# Autodesk Inventor assembly: assembly_camera
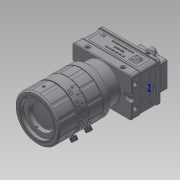
[picture p0: Inventor's stored thumbnail of the model, 180x180]
Saved by Autodesk Inventor 2017 (Build 210142000, 142)
## iProperties
Part Number: assembly_camera
Material: Generisch
Document SubType Name: Assembly
Designer: Max
Author: Max
## Documents named in this file (3)
- C:\Users\Max\Desktop\SENAI\robot_arm_new\assembly_camera.iam
- C:\Users\Max\Desktop\SENAI\robot_arm_new\EdmundOptics_lens.ipt
- C:\Users\Max\Desktop\SENAI\robot_arm_new\Genie-Nano-Sony_C-mount.ipt
## Components (2 placed, 2 different names)
1. EdmundOptics_lens:1 — Passend:1, Passend:2
2. Genie-Nano-Sony_C-mount:1 — Passend:1, Passend:2
## Relationships (2: Mate 2)
- Passend:1 [Mate]: EdmundOptics_lens:1 ↔ Genie-Nano-Sony_C-mount:1
- Passend:2 [Mate]: EdmundOptics_lens:1 ↔ Genie-Nano-Sony_C-mount:1
